# Autodesk Inventor assembly: Robot_arm
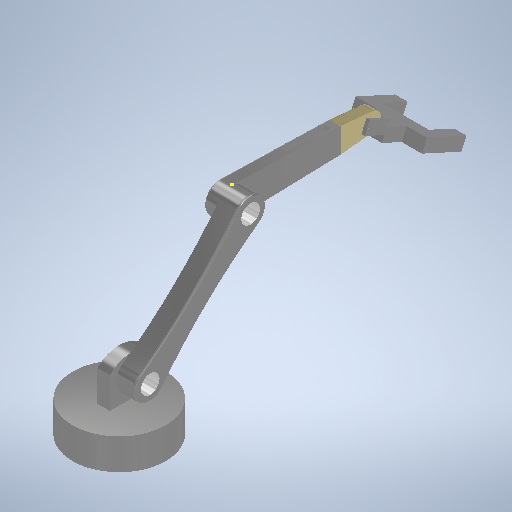
[picture p0: Inventor's stored thumbnail of the model, 512x512]
Saved by Autodesk Inventor 2025 (Build 290162010, 162A)
## iProperties
Created: 2024-07-13
Part Number: Robot_arm
Document SubType Name: Assembly
Designer: saees
Author: saees
## Documents named in this file (6)
- C:\Users\saees\OneDrive\Documents\Inventor\Robot_arm.iam
- C:\Users\saees\OneDrive\Documents\Inventor\Robot_arm_base.ipt
- C:\Users\saees\OneDrive\Documents\Inventor\Robot_arm_1.ipt
- C:\Users\saees\OneDrive\Documents\Inventor\Robot_arm_2.ipt
- C:\Users\saees\OneDrive\Documents\Inventor\Robot_arm_3.ipt
- C:\Users\saees\OneDrive\Documents\Inventor\Robot_arm_gripper.ipt
## Components (5 placed, 5 different names)
1. Robot_arm_base:1 — Mate:1, Mate:2, Mate:3
2. Robot_arm_1:1 — Mate:1, Mate:2, Mate:3, Mate:4, Mate:5
3. Robot_arm_2:1 — Mate:4, Mate:5, Mate:6, Flush:1, Mate:7
4. Robot_arm_3:1 — Mate:6, Flush:1, Mate:7, Mate:8, Mate:9
5. Robot_arm_gripper:1 — Mate:8, Mate:9
## Relationships (10: Mate 9, Flush 1)
- Mate:1: Robot_arm_base:1 ↔ Robot_arm_1:1
- Mate:2: Robot_arm_base:1 ↔ Robot_arm_1:1
- Mate:3: Robot_arm_base:1 ↔ Robot_arm_1:1
- Mate:4: Robot_arm_1:1 ↔ Robot_arm_2:1
- Mate:5: Robot_arm_1:1 ↔ Robot_arm_2:1
- Mate:6: Robot_arm_2:1 ↔ Robot_arm_3:1
- Flush:1: Robot_arm_2:1 ↔ Robot_arm_3:1
- Mate:7: Robot_arm_2:1 ↔ Robot_arm_3:1
- Mate:8: Robot_arm_3:1 ↔ Robot_arm_gripper:1
- Mate:9: Robot_arm_3:1 ↔ Robot_arm_gripper:1
